# Autodesk Inventor assembly: Assem_For_Print
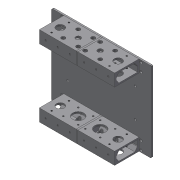
[picture p0: Inventor's stored thumbnail of the model, 180x180]
Saved by Autodesk Inventor 2018 (Build 220112000, 112)
## iProperties
Created: 2019-09-01
Part Number: Assem_For_Print
Document SubType Name: Assembly
Designer: Clevo
Author: Clevo
## Documents named in this file (5)
- E:\Hardware_Accelerated_Robot\Hardware\CustomParts\Assem_For_Print.iam
- E:\Hardware_Accelerated_Robot\Hardware\CustomParts\Battery_Base_ForPrint.ipt
- E:\Hardware_Accelerated_Robot\Hardware\CustomParts\Transmission_Case_ForPrint.ipt
- E:\Hardware_Accelerated_Robot\Hardware\CustomParts\Transmission_Case_ForPrint_MIR.ipt
- E:\Hardware_Accelerated_Robot\Hardware\CustomParts\Chassis_Spacer_ForPrint.ipt
## Components (7 placed, 4 different names)
1. Battery_Base_ForPrint:1 — Mate:1, Mate:2, Mate:3, Mate:4, Mate:5, Mate:6, Mate:7, Mate:8, Mate:9, Mate:10, Mate:11, Mate:12, Mate:13, Mate:15
2. Transmission_Case_ForPrint:1 — Mate:2, Mate:5, Mate:6, Mate:14
3. Transmission_Case_ForPrint:2 — Mate:1, Mate:3, Mate:4, Flush:2
4. Transmission_Case_ForPrint_MIR:1 — Mate:8, Mate:9, Mate:10, Mate:16
5. Transmission_Case_ForPrint_MIR:2 — Mate:7, Mate:11, Mate:12, Flush:1
6. Chassis_Spacer_ForPrint:1 — Mate:15, Flush:2, Mate:16
7. Chassis_Spacer_ForPrint:2 — Mate:13, Flush:1, Mate:14
## Relationships (18: Mate 16, Flush 2)
- Mate:1: Battery_Base_ForPrint:1 ↔ Transmission_Case_ForPrint:2
- Mate:2: Battery_Base_ForPrint:1 ↔ Transmission_Case_ForPrint:1
- Mate:3: Battery_Base_ForPrint:1 ↔ Transmission_Case_ForPrint:2
- Mate:4: Battery_Base_ForPrint:1 ↔ Transmission_Case_ForPrint:2
- Mate:5: Battery_Base_ForPrint:1 ↔ Transmission_Case_ForPrint:1
- Mate:6: Battery_Base_ForPrint:1 ↔ Transmission_Case_ForPrint:1
- Mate:7: Battery_Base_ForPrint:1 ↔ Transmission_Case_ForPrint_MIR:2
- Mate:8: Battery_Base_ForPrint:1 ↔ Transmission_Case_ForPrint_MIR:1
- Mate:9: Battery_Base_ForPrint:1 ↔ Transmission_Case_ForPrint_MIR:1
- Mate:10: Battery_Base_ForPrint:1 ↔ Transmission_Case_ForPrint_MIR:1
- Mate:11: Battery_Base_ForPrint:1 ↔ Transmission_Case_ForPrint_MIR:2
- Mate:12: Battery_Base_ForPrint:1 ↔ Transmission_Case_ForPrint_MIR:2
- Mate:13: Battery_Base_ForPrint:1 ↔ Chassis_Spacer_ForPrint:2
- Flush:1: Transmission_Case_ForPrint_MIR:2 ↔ Chassis_Spacer_ForPrint:2
- Mate:14: Transmission_Case_ForPrint:1 ↔ Chassis_Spacer_ForPrint:2
- Mate:15: Battery_Base_ForPrint:1 ↔ Chassis_Spacer_ForPrint:1
- Flush:2: Transmission_Case_ForPrint:2 ↔ Chassis_Spacer_ForPrint:1
- Mate:16: Transmission_Case_ForPrint_MIR:1 ↔ Chassis_Spacer_ForPrint:1
